# Autodesk Inventor assembly: Assembly_XY2_改
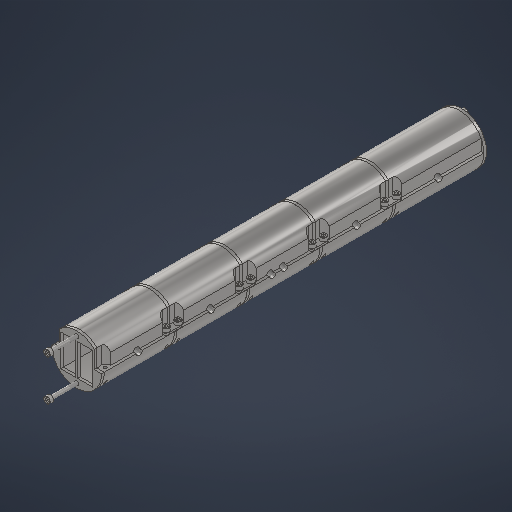
[picture p0: Inventor's stored thumbnail of the model, 512x512]
Saved by Autodesk Inventor 2026 (Build 300175050, 175E)
## iProperties
Created: 2026-02-23
Part Number: Assembly_XY2_改
Document SubType Name: Assembly
Designer: hirotaka-honda
Author: hirotaka-honda
## Documents named in this file (11)
- C:\Users\hirotaka-honda\Documents\HONDA\探索\触媒\カートリッジ触媒(波板+平板)\Φ54.5\カートリッジ試作\Assembly_全体_Φ54.5.iam
- C:\Users\hirotaka-honda\Documents\HONDA\探索\触媒\カートリッジ触媒(波板+平板)\Φ54.5\カートリッジ試作\A1_円筒_両切欠き＋片ネジ_Φ54.5.ipt
- C:\Users\hirotaka-honda\Documents\HONDA\探索\触媒\カートリッジ触媒(波板+平板)\Φ54.5\カートリッジ試作\C1_円板_切欠きあり＋スリットあり＋ネジなし_Φ54.5.ipt
- C:\Users\hirotaka-honda\Documents\HONDA\探索\触媒\カートリッジ触媒(波板+平板)\Φ54.5\カートリッジ試作\F_円筒_片切欠き＋両ネジ_100㎜_Φ54.5_M4あり.ipt
- C:\Users\hirotaka-honda\Documents\HONDA\探索\触媒\カートリッジ触媒(波板+平板)\Φ54.5\カートリッジ試作\D_円板_切欠きなし＋スリットなし＋ネジなし_Φ54.5_M4ボルト穴.ipt
- C:\Users\hirotaka-honda\Documents\HONDA\探索\触媒\カートリッジ触媒(波板+平板)\Φ54.5\カートリッジ試作\E_Plate_改_Φ54.5.ipt
- C:\ProgramData\Autodesk\Inventor 2026\Content Center\Libraries\ja-JP\JIS B 1176\JIS B 1176 - M4 x 8 - 0.7.ipt
- C:\Users\hirotaka-honda\Documents\HONDA\探索\触媒\カートリッジ触媒(波板+平板)\Φ54.5\カートリッジ試作\A2_円筒_両切欠き＋両ネジ_Φ54.5_側面穴2つ.ipt
- C:\Users\hirotaka-honda\Documents\HONDA\探索\触媒\カートリッジ触媒(波板+平板)\Φ54.5\カートリッジ試作\A3_円筒_両切欠き＋片ネジ_Φ54.5_M4あり.ipt
- C:\ProgramData\Autodesk\Inventor 2026\Content Center\Libraries\ja-JP\JIS B 1176\JIS B 1176 - M4 x 40 - 0.7.ipt
- C:\Users\hirotaka-honda\Documents\HONDA\探索\触媒\カートリッジ触媒(波板+平板)\Φ54.5\カートリッジ試作\C2_円板_切欠きあり＋スリットあり＋ネジなし_Φ54.5_M4ボルト穴.ipt
## Components (39 placed, 10 different names)
1. A3_円筒_両切欠き＋片ネジ_Φ54.5_M4あり:1 — 挿入:1, 挿入:2, 挿入:13, 挿入:41, メイト:24, メイト:26, メイト:28
2. A1_円筒_両切欠き＋片ネジ_Φ54.5:2 — 挿入:3, 挿入:4, 挿入:14, 挿入:17, 挿入:38, 挿入:42
3. A2_円筒_両切欠き＋両ネジ_Φ54.5_側面穴2つ:1 — 挿入:5, 挿入:6, 挿入:18, 挿入:21, 挿入:34, 挿入:37
4. A1_円筒_両切欠き＋片ネジ_Φ54.5:4 — 挿入:7, 挿入:8, 挿入:22, 挿入:25, 挿入:30, 挿入:33
5. F_円筒_片切欠き＋両ネジ_100㎜_Φ54.5_M4あり:1 — 挿入:9, 挿入:10, 挿入:26, 挿入:29, メイト:17, メイト:18
6. C2_円板_切欠きあり＋スリットあり＋ネジなし_Φ54.5_M4ボルト穴:1 — 挿入:1, メイト:23, メイト:26, メイト:27
7. C1_円板_切欠きあり＋スリットあり＋ネジなし_Φ54.5:2 — 挿入:2, 挿入:3
8. C1_円板_切欠きあり＋スリットあり＋ネジなし_Φ54.5:3 — 挿入:4, 挿入:5
9. C1_円板_切欠きあり＋スリットあり＋ネジなし_Φ54.5:4 — 挿入:6, 挿入:7
10. C1_円板_切欠きあり＋スリットあり＋ネジなし_Φ54.5:5 — 挿入:8, 挿入:9, メイト:17
11. D_円板_切欠きなし＋スリットなし＋ネジなし_Φ54.5_M4ボルト穴:1 — 挿入:10, メイト:18, メイト:19, メイト:20, メイト:21, メイト:22
12. E_Plate_改_Φ54.5:1 — メイト:1, 挿入:11, メイト:2, 挿入:12, 挿入:13, 挿入:14
13. JIS B 1176 - メートル M4 x 8:1 — メイト:1, 挿入:11
14. JIS B 1176 - メートル M4 x 8:2 — メイト:2, 挿入:12
15. E_Plate_改_Φ54.5:2 — 挿入:17, 挿入:18
16. JIS B 1176 - メートル M4 x 8:3
17. JIS B 1176 - メートル M4 x 8:4
18. E_Plate_改_Φ54.5:3 — 挿入:21, 挿入:22
19. JIS B 1176 - メートル M4 x 8:5
20. JIS B 1176 - メートル M4 x 8:6
21. E_Plate_改_Φ54.5:4 — 挿入:25, 挿入:26
22. JIS B 1176 - メートル M4 x 8:7
23. JIS B 1176 - メートル M4 x 8:8
24. E_Plate_改_Φ54.5:5 — 挿入:29, 挿入:30
25. JIS B 1176 - メートル M4 x 8:9
26. JIS B 1176 - メートル M4 x 8:10
27. E_Plate_改_Φ54.5:6 — 挿入:33, 挿入:34
28. JIS B 1176 - メートル M4 x 8:11
29. JIS B 1176 - メートル M4 x 8:12
30. E_Plate_改_Φ54.5:7 — 挿入:37, 挿入:38
31. JIS B 1176 - メートル M4 x 8:13
32. JIS B 1176 - メートル M4 x 8:14
33. E_Plate_改_Φ54.5:8 — 挿入:41, 挿入:42
34. JIS B 1176 - メートル M4 x 8:15
35. JIS B 1176 - メートル M4 x 8:16
36. JIS B 1176 - メートル M4 x 8:17 — メイト:19, メイト:20
37. JIS B 1176 - メートル M4 x 8:18 — メイト:21, メイト:22
38. JIS B 1176 - メートル M4 x 40:1 — メイト:23, メイト:24
39. JIS B 1176 - メートル M4 x 40:2 — メイト:27, メイト:28
## Relationships (69: Insert 42, Mate 27)
- 挿入:1 [Insert]: A3_円筒_両切欠き＋片ネジ_Φ54.5_M4あり:1 ↔ C2_円板_切欠きあり＋スリットあり＋ネジなし_Φ54.5_M4ボルト穴:1
- 挿入:2 [Insert]: A3_円筒_両切欠き＋片ネジ_Φ54.5_M4あり:1 ↔ C1_円板_切欠きあり＋スリットあり＋ネジなし_Φ54.5:2
- 挿入:3 [Insert]: A1_円筒_両切欠き＋片ネジ_Φ54.5:2 ↔ C1_円板_切欠きあり＋スリットあり＋ネジなし_Φ54.5:2
- 挿入:4 [Insert]: A1_円筒_両切欠き＋片ネジ_Φ54.5:2 ↔ C1_円板_切欠きあり＋スリットあり＋ネジなし_Φ54.5:3
- 挿入:5 [Insert]: A2_円筒_両切欠き＋両ネジ_Φ54.5_側面穴2つ:1 ↔ C1_円板_切欠きあり＋スリットあり＋ネジなし_Φ54.5:3
- 挿入:6 [Insert]: A2_円筒_両切欠き＋両ネジ_Φ54.5_側面穴2つ:1 ↔ C1_円板_切欠きあり＋スリットあり＋ネジなし_Φ54.5:4
- 挿入:7 [Insert]: A1_円筒_両切欠き＋片ネジ_Φ54.5:4 ↔ C1_円板_切欠きあり＋スリットあり＋ネジなし_Φ54.5:4
- 挿入:8 [Insert]: A1_円筒_両切欠き＋片ネジ_Φ54.5:4 ↔ C1_円板_切欠きあり＋スリットあり＋ネジなし_Φ54.5:5
- 挿入:9 [Insert]: F_円筒_片切欠き＋両ネジ_100㎜_Φ54.5_M4あり:1 ↔ C1_円板_切欠きあり＋スリットあり＋ネジなし_Φ54.5:5
- 挿入:10 [Insert]: F_円筒_片切欠き＋両ネジ_100㎜_Φ54.5_M4あり:1 ↔ D_円板_切欠きなし＋スリットなし＋ネジなし_Φ54.5_M4ボルト穴:1
- メイト:1 [Mate]: E_Plate_改_Φ54.5:1 ↔ JIS B 1176 - メートル M4 x 8:1
- 挿入:11 [Insert]: E_Plate_改_Φ54.5:1 ↔ JIS B 1176 - メートル M4 x 8:1
- メイト:2 [Mate]: E_Plate_改_Φ54.5:1 ↔ JIS B 1176 - メートル M4 x 8:2
- 挿入:12 [Insert]: E_Plate_改_Φ54.5:1 ↔ JIS B 1176 - メートル M4 x 8:2
- 挿入:13 [Insert]: A3_円筒_両切欠き＋片ネジ_Φ54.5_M4あり:1 ↔ E_Plate_改_Φ54.5:1
- 挿入:14 [Insert]: A1_円筒_両切欠き＋片ネジ_Φ54.5:2 ↔ E_Plate_改_Φ54.5:1
- [Mate]: E_Plate_改_Φ54.5:2 ↔ JIS B 1176 - メートル M4 x 8:3
- [Insert]: E_Plate_改_Φ54.5:2 ↔ JIS B 1176 - メートル M4 x 8:3
- [Mate]: E_Plate_改_Φ54.5:2 ↔ JIS B 1176 - メートル M4 x 8:4
- [Insert]: E_Plate_改_Φ54.5:2 ↔ JIS B 1176 - メートル M4 x 8:4
- 挿入:17 [Insert]: A1_円筒_両切欠き＋片ネジ_Φ54.5:2 ↔ E_Plate_改_Φ54.5:2
- 挿入:18 [Insert]: A2_円筒_両切欠き＋両ネジ_Φ54.5_側面穴2つ:1 ↔ E_Plate_改_Φ54.5:2
- [Mate]: E_Plate_改_Φ54.5:3 ↔ JIS B 1176 - メートル M4 x 8:5
- [Insert]: E_Plate_改_Φ54.5:3 ↔ JIS B 1176 - メートル M4 x 8:5
- [Mate]: E_Plate_改_Φ54.5:3 ↔ JIS B 1176 - メートル M4 x 8:6
- [Insert]: E_Plate_改_Φ54.5:3 ↔ JIS B 1176 - メートル M4 x 8:6
- 挿入:21 [Insert]: A2_円筒_両切欠き＋両ネジ_Φ54.5_側面穴2つ:1 ↔ E_Plate_改_Φ54.5:3
- 挿入:22 [Insert]: A1_円筒_両切欠き＋片ネジ_Φ54.5:4 ↔ E_Plate_改_Φ54.5:3
- [Mate]: E_Plate_改_Φ54.5:4 ↔ JIS B 1176 - メートル M4 x 8:7
- [Insert]: E_Plate_改_Φ54.5:4 ↔ JIS B 1176 - メートル M4 x 8:7
- [Mate]: E_Plate_改_Φ54.5:4 ↔ JIS B 1176 - メートル M4 x 8:8
- [Insert]: E_Plate_改_Φ54.5:4 ↔ JIS B 1176 - メートル M4 x 8:8
- 挿入:25 [Insert]: A1_円筒_両切欠き＋片ネジ_Φ54.5:4 ↔ E_Plate_改_Φ54.5:4
- 挿入:26 [Insert]: F_円筒_片切欠き＋両ネジ_100㎜_Φ54.5_M4あり:1 ↔ E_Plate_改_Φ54.5:4
- [Mate]: E_Plate_改_Φ54.5:5 ↔ JIS B 1176 - メートル M4 x 8:9
- [Insert]: E_Plate_改_Φ54.5:5 ↔ JIS B 1176 - メートル M4 x 8:9
- [Mate]: E_Plate_改_Φ54.5:5 ↔ JIS B 1176 - メートル M4 x 8:10
- [Insert]: E_Plate_改_Φ54.5:5 ↔ JIS B 1176 - メートル M4 x 8:10
- 挿入:29 [Insert]: F_円筒_片切欠き＋両ネジ_100㎜_Φ54.5_M4あり:1 ↔ E_Plate_改_Φ54.5:5
- 挿入:30 [Insert]: A1_円筒_両切欠き＋片ネジ_Φ54.5:4 ↔ E_Plate_改_Φ54.5:5
- [Mate]: E_Plate_改_Φ54.5:6 ↔ JIS B 1176 - メートル M4 x 8:11
- [Insert]: E_Plate_改_Φ54.5:6 ↔ JIS B 1176 - メートル M4 x 8:11
- [Mate]: E_Plate_改_Φ54.5:6 ↔ JIS B 1176 - メートル M4 x 8:12
- [Insert]: E_Plate_改_Φ54.5:6 ↔ JIS B 1176 - メートル M4 x 8:12
- 挿入:33 [Insert]: A1_円筒_両切欠き＋片ネジ_Φ54.5:4 ↔ E_Plate_改_Φ54.5:6
- 挿入:34 [Insert]: A2_円筒_両切欠き＋両ネジ_Φ54.5_側面穴2つ:1 ↔ E_Plate_改_Φ54.5:6
- [Mate]: E_Plate_改_Φ54.5:7 ↔ JIS B 1176 - メートル M4 x 8:13
- [Insert]: E_Plate_改_Φ54.5:7 ↔ JIS B 1176 - メートル M4 x 8:13
- [Mate]: E_Plate_改_Φ54.5:7 ↔ JIS B 1176 - メートル M4 x 8:14
- [Insert]: E_Plate_改_Φ54.5:7 ↔ JIS B 1176 - メートル M4 x 8:14
- 挿入:37 [Insert]: A2_円筒_両切欠き＋両ネジ_Φ54.5_側面穴2つ:1 ↔ E_Plate_改_Φ54.5:7
- 挿入:38 [Insert]: A1_円筒_両切欠き＋片ネジ_Φ54.5:2 ↔ E_Plate_改_Φ54.5:7
- [Mate]: E_Plate_改_Φ54.5:8 ↔ JIS B 1176 - メートル M4 x 8:15
- [Insert]: E_Plate_改_Φ54.5:8 ↔ JIS B 1176 - メートル M4 x 8:15
- [Mate]: E_Plate_改_Φ54.5:8 ↔ JIS B 1176 - メートル M4 x 8:16
- [Insert]: E_Plate_改_Φ54.5:8 ↔ JIS B 1176 - メートル M4 x 8:16
- 挿入:41 [Insert]: A3_円筒_両切欠き＋片ネジ_Φ54.5_M4あり:1 ↔ E_Plate_改_Φ54.5:8
- 挿入:42 [Insert]: A1_円筒_両切欠き＋片ネジ_Φ54.5:2 ↔ E_Plate_改_Φ54.5:8
- メイト:17 [Mate]: F_円筒_片切欠き＋両ネジ_100㎜_Φ54.5_M4あり:1 ↔ C1_円板_切欠きあり＋スリットあり＋ネジなし_Φ54.5:5
- メイト:18 [Mate]: F_円筒_片切欠き＋両ネジ_100㎜_Φ54.5_M4あり:1 ↔ D_円板_切欠きなし＋スリットなし＋ネジなし_Φ54.5_M4ボルト穴:1
- メイト:19 [Mate]: D_円板_切欠きなし＋スリットなし＋ネジなし_Φ54.5_M4ボルト穴:1 ↔ JIS B 1176 - メートル M4 x 8:17
- メイト:20 [Mate]: D_円板_切欠きなし＋スリットなし＋ネジなし_Φ54.5_M4ボルト穴:1 ↔ JIS B 1176 - メートル M4 x 8:17
- メイト:21 [Mate]: D_円板_切欠きなし＋スリットなし＋ネジなし_Φ54.5_M4ボルト穴:1 ↔ JIS B 1176 - メートル M4 x 8:18
- メイト:22 [Mate]: D_円板_切欠きなし＋スリットなし＋ネジなし_Φ54.5_M4ボルト穴:1 ↔ JIS B 1176 - メートル M4 x 8:18
- メイト:23 [Mate]: C2_円板_切欠きあり＋スリットあり＋ネジなし_Φ54.5_M4ボルト穴:1 ↔ JIS B 1176 - メートル M4 x 40:1
- メイト:24 [Mate] (8 mm): A3_円筒_両切欠き＋片ネジ_Φ54.5_M4あり:1 ↔ JIS B 1176 - メートル M4 x 40:1
- メイト:26 [Mate]: A3_円筒_両切欠き＋片ネジ_Φ54.5_M4あり:1 ↔ C2_円板_切欠きあり＋スリットあり＋ネジなし_Φ54.5_M4ボルト穴:1
- メイト:27 [Mate]: C2_円板_切欠きあり＋スリットあり＋ネジなし_Φ54.5_M4ボルト穴:1 ↔ JIS B 1176 - メートル M4 x 40:2
- メイト:28 [Mate] (-8 mm): A3_円筒_両切欠き＋片ネジ_Φ54.5_M4あり:1 ↔ JIS B 1176 - メートル M4 x 40:2
## Named parameters: d104_d99 = 0 mm, d105_d100 = 0 mm, d106_d101 = 0 mm, d107_d98 = 0 mm, d110_d104_d99 = 0 mm, d111_d105_d100 = 0 mm, d112_d106_d101 = 0 mm, d113_d107_d98 = 0 mm, d116_d104_d99 = 0 mm, d117_d105_d100 = 0 mm, d118_d106_d101 = 0 mm, d119_d107_d98 = 0 mm, d122_d104_d99 = 0 mm, d123_d105_d100 = 0 mm, d124_d106_d101 = 0 mm, d125_d107_d98 = 0 mm, d128_d104_d99 = 0 mm, d129_d105_d100 = 0 mm, d130_d106_d101 = 0 mm, d131_d107_d98 = 0 mm, d134_d104_d99 = 0 mm, d135_d105_d100 = 0 mm, d136_d106_d101 = 0 mm, d137_d107_d98 = 0 mm, d140_d104_d99 = 0 mm, d141_d105_d100 = 0 mm, d142_d106_d101 = 0 mm, d143_d107_d98 = 0 mm
